# Autodesk Inventor assembly: Base
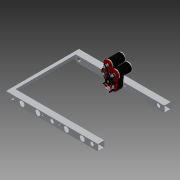
[picture p0: Inventor's stored thumbnail of the model, 180x180]
Saved by Autodesk Inventor 2013 (Build 170138000, 138)
## iProperties
Created: 2013-09-20
Part Number: Base
Document SubType Name: Assembly
Designer: grtstudent
Author: grtstudent
## Documents named in this file (5)
- C:\Users\grtstudent\Desktop\Final Preseason\Base (2013)\Base.iam
- C:\Users\grtstudent\Desktop\Final Preseason\Base (2013)\LeftMainBeam.ipt
- C:\Users\grtstudent\Desktop\Final Preseason\Base (2013)\RightMainBeam.ipt
- C:\Users\grtstudent\Desktop\Final Preseason\Base (2013)\End Beam.ipt
- C:\Users\grtstudent\Desktop\Final Preseason\Mark 6 - Final Preseason.iam
## Components (4 placed, 4 different names)
1. LeftMainBeam:1 — Mate:1, Mate:2, Mate:4, Mate:5, Mate:6, Mate:7
2. RightMainBeam:1 — Mate:1, Mate:2, Flush:1, Mate:2, Mate:3
3. End Beam:1 — Flush:1, Mate:2, Mate:3, Mate:4
4. Mark 6 - Final Preseason:1 [sub-assembly] — Mate:5, Mate:6, Mate:7
## Relationships (9: Mate 8, Flush 1)
- Mate:1: LeftMainBeam:1 ↔ RightMainBeam:1
- Mate:2: LeftMainBeam:1 ↔ RightMainBeam:1
- Flush:1: RightMainBeam:1 ↔ End Beam:1
- Mate:2: RightMainBeam:1 ↔ End Beam:1
- Mate:3: RightMainBeam:1 ↔ End Beam:1
- Mate:4: LeftMainBeam:1 ↔ End Beam:1
- Mate:5: LeftMainBeam:1 ↔ Mark 6 - Final Preseason:1
- Mate:6: LeftMainBeam:1 ↔ Mark 6 - Final Preseason:1
- Mate:7: LeftMainBeam:1 ↔ Mark 6 - Final Preseason:1
